# Autodesk Inventor assembly: 1210 ASY GBK long wall shield 3
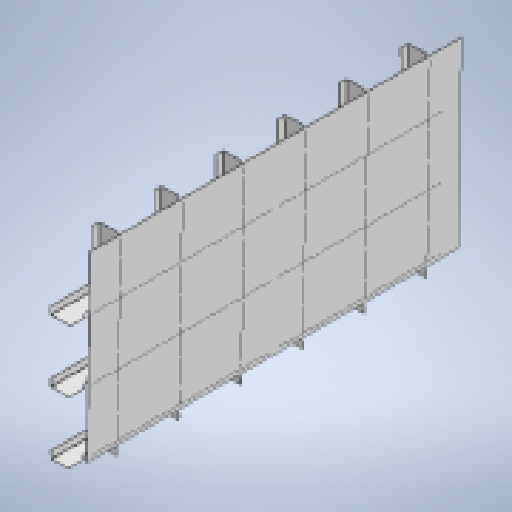
[picture p0: Inventor's stored thumbnail of the model, 512x512]
Saved by Autodesk Inventor 2026.2 (Build 302298000, 298)
## iProperties
Created: 2026-05-07
Part Number: 1210 ASY GBK long wall shield 3
Document SubType Name: Assembly
Designer: pokla
Mass: 252568 g
Surface Area: 163192 cm^2
Volume: 32174.3 cm^3
Density: 7.85 g/cm^3
Author: admin
## Documents named in this file (7)
- C:\Users\admin\Documents\Inventor\GBK-Gubkinskiy\04 ASY GBK wall shield 1.2.4.iam
- C:\Users\admin\Documents\Inventor\GBK-Gubkinskiy\0241 GBK shield 4.ipt
- C:\Users\admin\Documents\Inventor\GBK-Gubkinskiy\04.2 GBK rib.ipt
- C:\Users\admin\Documents\Inventor\GBK-Gubkinskiy\0241 GBK stringer 4.ipt
- C:\Users\admin\Documents\Inventor\GBK-Gubkinskiy\0242 GBK stringer 5.ipt
- C:\Users\admin\Documents\Inventor\GBK-Gubkinskiy\0243 GBK stringer 6.ipt
- C:\Users\admin\Documents\Inventor\GBK-Gubkinskiy\01.2 GBK main rib.ipt
## Components (13 placed, 5 different names)
1. 0241 GBK stringer 4:1
2. 0241 GBK stringer 4:2
3. 0242 GBK stringer 5:1
4. 0242 GBK stringer 5:2
5. 0243 GBK stringer 6:1
6. 0243 GBK stringer 6:2
7. 0241 GBK shield 4:1
8. 04.2 GBK rib:1
9. 04.2 GBK rib:2
10. 04.2 GBK rib:3
11. 04.2 GBK rib:4
12. 04.2 GBK rib:5
13. 04.2 GBK rib:6
## Component patterns: (6 elements, first: 04.2 GBK rib:1)
## Relationships (9: WeldJoint 6, Mate 2, Flush 1)
- [Flush] (250 mm): 0241 GBK shield 4:1 ↔ 04.2 GBK rib:1
- [Mate]: 0241 GBK shield 4:1 ↔ 04.2 GBK rib:1
- [Mate]: 0241 GBK shield 4:1 ↔ 04.2 GBK rib:1
- [WeldJoint]: 0241 GBK stringer 4:1 ↔ 0241 GBK stringer 4:2
- [WeldJoint]: 0242 GBK stringer 5:1 ↔ 0242 GBK stringer 5:2
- [WeldJoint]: 0243 GBK stringer 6:1 ↔ 0243 GBK stringer 6:2
- [WeldJoint] (4 mm): 0243 GBK stringer 6:1 ↔ 04.2 GBK rib:1
- [WeldJoint] (4 mm): 0242 GBK stringer 5:1 ↔ 04.2 GBK rib:1
- [WeldJoint] (4 mm): 0241 GBK stringer 4:1 ↔ 04.2 GBK rib:1
## Named parameters: Шаг_шпангоутов = 496.66667 mm
